# Autodesk Inventor assembly: DE_assembly_Ocampo
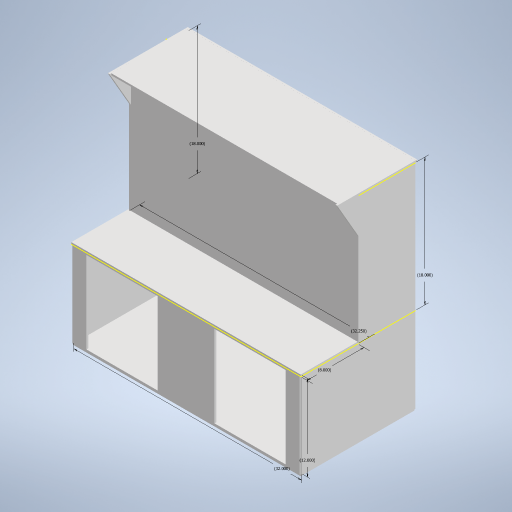
[picture p0: Inventor's stored thumbnail of the model, 512x512]
Saved by Autodesk Inventor 2023 (Build 270158000, 158)
## iProperties
Created: 2025-02-18
Part Number: DE_assembly_Ocampo
Document SubType Name: Assembly
Designer: 1244275
Author: 1244275
## Documents named in this file (10)
- G:\My Drive\Digital Electronics\DE_assembly_Ocampo.iam
- G:\My Drive\Digital Electronics\bottom_bottom_plywood_Ocampo.ipt
- G:\My Drive\Digital Electronics\side_bottom_plywood_Ocampo.ipt
- G:\My Drive\Digital Electronics\bottom_plywood_Ocampo.ipt
- G:\My Drive\Digital Electronics\top_top_plywood_Ocampo.ipt
- G:\My Drive\Digital Electronics\side_top_plywood_Ocampo.ipt
- G:\My Drive\Digital Electronics\triangle_plywood_Ocampo.ipt
- G:\My Drive\Digital Electronics\half_top_plywood_Ocampo.ipt
- G:\My Drive\Digital Electronics\big_back_plywood_Ocampo.ipt
- G:\My Drive\Digital Electronics\top_plywood_Ocampo.ipt
## Components (12 placed, 9 different names)
1. bottom_bottom_plywood_Ocampo:1 — Flush:1, Rigid:1, Flush:2, Rigid:2, Rigid:3
2. side_bottom_plywood_Ocampo:1 — Flush:1, Rigid:1, Mate:1, Mate:4, Flush:7, Flush:8
3. side_bottom_plywood_Ocampo:2 — Flush:2, Rigid:2, Mate:3, Flush:5, Flush:6, Mate:8, Flush:17
4. bottom_plywood_Ocampo:1 — Mate:1, Rigid:3, Flush:16
5. side_top_plywood_Ocampo:1 — Mate:3, Flush:5, Flush:6, Mate:6, Flush:12, Mate:9, Flush:18, Mate:10, Flush:20, Flush:22
6. side_top_plywood_Ocampo:2 — Mate:4, Flush:7, Flush:8, Mate:7, Flush:14, Mate:11
7. triangle_plywood_Ocampo:1 — Mate:6, Flush:12
8. triangle_plywood_Ocampo:2 — Mate:7, Flush:14
9. half_top_plywood_Ocampo:1 — Mate:8, Flush:16, Flush:17
10. big_back_plywood_Ocampo:1 — Mate:9, Flush:18, Flush:21
11. top_plywood_Ocampo:1 — Mate:10, Flush:20, Mate:12
12. top_top_plywood_Ocampo:1 — Mate:11, Flush:21, Flush:22, Mate:12
## Relationships (27: Flush 14, Mate 10, WeldJoint 3)
- Flush:1: bottom_bottom_plywood_Ocampo:1 ↔ side_bottom_plywood_Ocampo:1
- Rigid:1 [WeldJoint]: bottom_bottom_plywood_Ocampo:1 ↔ side_bottom_plywood_Ocampo:1
- Flush:2: bottom_bottom_plywood_Ocampo:1 ↔ side_bottom_plywood_Ocampo:2
- Rigid:2 [WeldJoint]: bottom_bottom_plywood_Ocampo:1 ↔ side_bottom_plywood_Ocampo:2
- Mate:1: side_bottom_plywood_Ocampo:1 ↔ bottom_plywood_Ocampo:1
- Rigid:3 [WeldJoint]: bottom_bottom_plywood_Ocampo:1 ↔ bottom_plywood_Ocampo:1
- Mate:3: side_bottom_plywood_Ocampo:2 ↔ side_top_plywood_Ocampo:1
- Flush:5: side_bottom_plywood_Ocampo:2 ↔ side_top_plywood_Ocampo:1
- Flush:6: side_bottom_plywood_Ocampo:2 ↔ side_top_plywood_Ocampo:1
- Mate:4: side_bottom_plywood_Ocampo:1 ↔ side_top_plywood_Ocampo:2
- Flush:7: side_bottom_plywood_Ocampo:1 ↔ side_top_plywood_Ocampo:2
- Flush:8: side_bottom_plywood_Ocampo:1 ↔ side_top_plywood_Ocampo:2
- Mate:6: side_top_plywood_Ocampo:1 ↔ triangle_plywood_Ocampo:1
- Flush:12: side_top_plywood_Ocampo:1 ↔ triangle_plywood_Ocampo:1
- Mate:7: side_top_plywood_Ocampo:2 ↔ triangle_plywood_Ocampo:2
- Flush:14: side_top_plywood_Ocampo:2 ↔ triangle_plywood_Ocampo:2
- Mate:8: side_bottom_plywood_Ocampo:2 ↔ half_top_plywood_Ocampo:1
- Flush:16: bottom_plywood_Ocampo:1 ↔ half_top_plywood_Ocampo:1
- Flush:17: side_bottom_plywood_Ocampo:2 ↔ half_top_plywood_Ocampo:1
- Mate:9: side_top_plywood_Ocampo:1 ↔ big_back_plywood_Ocampo:1
- Flush:18: side_top_plywood_Ocampo:1 ↔ big_back_plywood_Ocampo:1
- Mate:10: side_top_plywood_Ocampo:1 ↔ top_plywood_Ocampo:1
- Flush:20: side_top_plywood_Ocampo:1 ↔ top_plywood_Ocampo:1
- Mate:11: side_top_plywood_Ocampo:2 ↔ top_top_plywood_Ocampo:1
- Flush:21: big_back_plywood_Ocampo:1 ↔ top_top_plywood_Ocampo:1
- Flush:22: side_top_plywood_Ocampo:1 ↔ top_top_plywood_Ocampo:1
- Mate:12: top_plywood_Ocampo:1 ↔ top_top_plywood_Ocampo:1
